# Autodesk Inventor assembly: Шкив+ подшипники
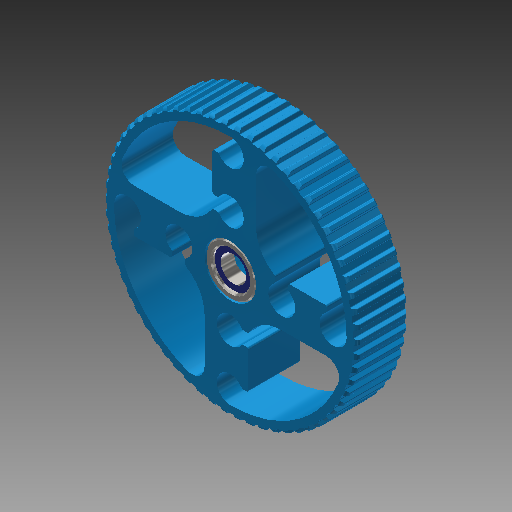
[picture p0: Inventor's stored thumbnail of the model, 512x512]
Saved by Autodesk Inventor 2019 (Build 230136000, 136)
## iProperties
Created: 2019-08-15
Part Number: Шкив+ подшипники
Material: Типовые
Document SubType Name: Assembly
Designer: Петров Иван
Author: Петров Иван
## Documents named in this file (3)
- C:\Users\user\Documents\Kvantoriada2019\optimal_gripper\hardware\Стандартные изделия\Шкив большой сборка.iam
- C:\Users\user\Documents\Kvantoriada2019\optimal_gripper\hardware\Стандартные изделия\Шкив большой Makeblock.ipt
- C:\Users\user\Documents\Kvantoriada2019\optimal_gripper\hardware\Стандартные изделия\Подшипник 4x8x3.ipt
## Components (3 placed, 2 different names)
1. Шкив большой Makeblock:1 — Совмещение:1, Заподлицо:1, Совмещение:2, Заподлицо:2
2. Подшипник 4x8x3:1 — Совмещение:1, Заподлицо:1
3. Подшипник 4x8x3:2 — Совмещение:2, Заподлицо:2
## Relationships (4: Mate 2, Flush 2)
- Совмещение:1 [Mate]: Шкив большой Makeblock:1 ↔ Подшипник 4x8x3:1
- Заподлицо:1 [Flush]: Шкив большой Makeblock:1 ↔ Подшипник 4x8x3:1
- Совмещение:2 [Mate]: Шкив большой Makeblock:1 ↔ Подшипник 4x8x3:2
- Заподлицо:2 [Flush]: Шкив большой Makeblock:1 ↔ Подшипник 4x8x3:2
